# Autodesk Inventor assembly: Back Electrical Board
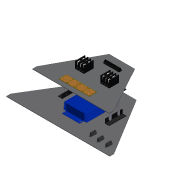
[picture p0: Inventor's stored thumbnail of the model, 180x180]
Saved by Autodesk Inventor 2012 (Build 160160000, 160)
## iProperties
Created: 2012-01-14
Part Number: Back Electrical Board
Document SubType Name: Assembly
Designer: Antonella Wilby
Author: Antonella Wilby
## Documents named in this file (8)
- C:\Users\Antonella\Documents\GCC Robotics 2012 - Mechanical\Robot 2.0\Electrical\Back Electrical Board\Back Electrical Board.iam
- C:\Users\Antonella\Documents\GCC Robotics 2012 - Mechanical\Robot 2.0\Electrical\Back Electrical Board\Bottom\Electrical Board - back bottom.iam
- C:\Users\Antonella\Documents\GCC Robotics 2012 - Mechanical\Robot 2.0\Electrical\Back Electrical Board\Top\Electrical Board - back top.iam
- C:\Users\Antonella\Documents\GCC Robotics 2012 - Mechanical\Robot 2.0\Electrical\Back Electrical Board\top bottom link.ipt
- C:\Users\Antonella\Documents\GCC Robotics 2012 - Mechanical\Robot 2.0\Other Models\DirectMountTerminalBlock_AutomationDirect_BM-M092CS.iam
- C:\Users\Antonella\Documents\GCC Robotics 2012 - Mechanical\Robot 2.0\Other Models\Mini Board\Mini Board.ipt
- C:\Users\Antonella\Documents\GCC Robotics 2012 - Mechanical\Robot 2.0\Other Models\Sharp Sensor\Sharp GP2Y0 Sensor.iam
- C:\Users\Antonella\Documents\GCC Robotics 2012 - Mechanical\Robot 2.0\Other Models\Power Block\Power Block.iam
## Components (16 placed, 7 different names)
1. Electrical Board - back bottom:1 [sub-assembly] — Mate:1, Mate:2, Mate:3, Mate:4, Mate:5, Mate:6, Mate:7, Mate:8, Flush:1, Mate:21, Flush:7, Flush:8, Mate:22, Mate:23, Flush:9
2. Electrical Board - back top:1 [sub-assembly] — Mate:9, Mate:10, Mate:11, Mate:12, Flush:1, Mate:13, Flush:2, Mate:14, Mate:15, Mate:17, Mate:19, Flush:6, Mate:24, Flush:10, Mate:25, Flush:11, Flush:12
3. top bottom link:1 — Mate:3, Mate:4, Mate:11
4. top bottom link:2 — Mate:1, Mate:2, Mate:12
5. top bottom link:3 — Mate:7, Mate:8, Mate:9
6. top bottom link:4 — Mate:5, Mate:6, Mate:10
7. DirectMountTerminalBlock_AutomationDirect_BM-M092CS:1 [sub-assembly] — Mate:13, Flush:2
8. Mini Board:1 — Mate:14, Mate:16, Flush:3, Flush:6
9. Mini Board:2 — Mate:15, Mate:16, Flush:3, Mate:18, Flush:4
10. Mini Board:3 — Mate:17, Mate:18, Flush:4, Flush:5, Mate:20
11. Mini Board:4 — Mate:19, Flush:5, Mate:20
12. Sharp GP2Y0 Sensor:1 [sub-assembly] — Mate:21, Flush:7
13. Sharp GP2Y0 Sensor:2 [sub-assembly] — Mate:23, Flush:9
14. Sharp GP2Y0 Sensor:3 [sub-assembly] — Flush:8, Mate:22
15. Power Block:1 [sub-assembly] — Mate:24, Flush:10, Flush:13
16. Power Block:2 [sub-assembly] — Mate:25, Flush:11, Flush:12, Flush:13
## Relationships (38: Mate 25, Flush 13)
- Mate:1: Electrical Board - back bottom:1 ↔ top bottom link:2
- Mate:2: Electrical Board - back bottom:1 ↔ top bottom link:2
- Mate:3: Electrical Board - back bottom:1 ↔ top bottom link:1
- Mate:4: Electrical Board - back bottom:1 ↔ top bottom link:1
- Mate:5: Electrical Board - back bottom:1 ↔ top bottom link:4
- Mate:6: Electrical Board - back bottom:1 ↔ top bottom link:4
- Mate:7: Electrical Board - back bottom:1 ↔ top bottom link:3
- Mate:8: Electrical Board - back bottom:1 ↔ top bottom link:3
- Mate:9: Electrical Board - back top:1 ↔ top bottom link:3
- Mate:10: Electrical Board - back top:1 ↔ top bottom link:4
- Mate:11: Electrical Board - back top:1 ↔ top bottom link:1
- Mate:12: Electrical Board - back top:1 ↔ top bottom link:2
- Flush:1: Electrical Board - back bottom:1 ↔ Electrical Board - back top:1
- Mate:13: Electrical Board - back top:1 ↔ DirectMountTerminalBlock_AutomationDirect_BM-M092CS:1
- Flush:2 (-50.8 mm): Electrical Board - back top:1 ↔ DirectMountTerminalBlock_AutomationDirect_BM-M092CS:1
- Mate:14: Electrical Board - back top:1 ↔ Mini Board:1
- Mate:15: Electrical Board - back top:1 ↔ Mini Board:2
- Mate:16: Mini Board:1 ↔ Mini Board:2
- Flush:3: Mini Board:1 ↔ Mini Board:2
- Mate:17: Electrical Board - back top:1 ↔ Mini Board:3
- Mate:18: Mini Board:2 ↔ Mini Board:3
- Flush:4: Mini Board:2 ↔ Mini Board:3
- Mate:19: Electrical Board - back top:1 ↔ Mini Board:4
- Flush:5: Mini Board:3 ↔ Mini Board:4
- Mate:20: Mini Board:3 ↔ Mini Board:4
- Flush:6 (25.4 mm): Electrical Board - back top:1 ↔ Mini Board:1
- Mate:21: Electrical Board - back bottom:1 ↔ Sharp GP2Y0 Sensor:1
- Flush:7 (50.8 mm): Electrical Board - back bottom:1 ↔ Sharp GP2Y0 Sensor:1
- Flush:8 (101.6 mm): Electrical Board - back bottom:1 ↔ Sharp GP2Y0 Sensor:3
- Mate:22: Electrical Board - back bottom:1 ↔ Sharp GP2Y0 Sensor:3
- Mate:23: Electrical Board - back bottom:1 ↔ Sharp GP2Y0 Sensor:2
- Flush:9 (152.4 mm): Electrical Board - back bottom:1 ↔ Sharp GP2Y0 Sensor:2
- Mate:24: Electrical Board - back top:1 ↔ Power Block:1
- Flush:10 (127 mm): Electrical Board - back top:1 ↔ Power Block:1
- Mate:25: Electrical Board - back top:1 ↔ Power Block:2
- Flush:11 (-127 mm): Electrical Board - back top:1 ↔ Power Block:2
- Flush:12 (-127 mm): Electrical Board - back top:1 ↔ Power Block:2
- Flush:13: Power Block:1 ↔ Power Block:2
